# Autodesk Inventor assembly: WedgeBotV1
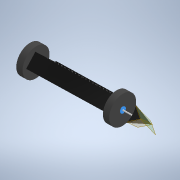
[picture p0: Inventor's stored thumbnail of the model, 180x180]
Saved by Autodesk Inventor 2020 (Build 240168000, 168)
## iProperties
Created: 2023-12-01
Part Number: WedgeBotV1
Document SubType Name: Assembly
Designer: smz3rm
Mass: 451.91 g
Surface Area: 928.874 cm^2
Volume: 362.181 cm^3
Density: 1.24775 g/cm^3
Author: smz3rm
## Documents named in this file (6)
- C:\Users\smz3rm\OneDrive - BP\Documents\DigitalTwin\Models\BattleBot\WedgeBotV1.iam
- C:\Users\smz3rm\OneDrive - BP\Documents\DigitalTwin\Models\BattleBot\DriveMotorV2.ipt
- C:\Users\smz3rm\OneDrive - BP\Documents\DigitalTwin\Models\BattleBot\HubV2.ipt
- C:\Users\smz3rm\OneDrive - BP\Documents\DigitalTwin\Models\BattleBot\WheelV1.ipt
- C:\Users\smz3rm\OneDrive - BP\Documents\DigitalTwin\Models\BattleBot\BodyWedgeV3.ipt
- C:\Users\smz3rm\OneDrive - BP\Documents\DigitalTwin\Models\BattleBot\BatteryV1.ipt
## Components (8 placed, 5 different names)
1. DriveMotorV2:1 — Mate:2, Mate:13, Mate:14, Mate:15
2. HubV2:1 — Cylindrical:1, Mate:1, Mate:2, Mate:21
3. WheelV1:1 — Cylindrical:1, Mate:1, Tangent:1
4. WheelV1:2 — Mate:7, Mate:8
5. DriveMotorV2:2 — Mate:9, Mate:10, Mate:11, Mate:12
6. HubV2:2 — Mate:7, Mate:8, Mate:9, Mate:20
7. BodyWedgeV3:1 — Mate:10, Mate:11, Mate:12, Mate:13, Mate:14, Mate:15, Mate:16, Mate:17, Mate:18, Mate:19, Mate:20, Mate:21
8. BatteryV1:1 — Mate:16, Mate:17, Mate:18
## Relationships (19: Mate 17, CylindricalJoint 1, Tangent 1)
- Cylindrical:1: HubV2:1 ↔ WheelV1:1
- Mate:1: HubV2:1 ↔ WheelV1:1
- Mate:2: DriveMotorV2:1 ↔ HubV2:1
- Mate:7: WheelV1:2 ↔ HubV2:2
- Mate:8: WheelV1:2 ↔ HubV2:2
- Mate:9: DriveMotorV2:2 ↔ HubV2:2
- Mate:10: DriveMotorV2:2 ↔ BodyWedgeV3:1
- Mate:11: DriveMotorV2:2 ↔ BodyWedgeV3:1
- Mate:12: DriveMotorV2:2 ↔ BodyWedgeV3:1
- Mate:13: DriveMotorV2:1 ↔ BodyWedgeV3:1
- Mate:14: DriveMotorV2:1 ↔ BodyWedgeV3:1
- Mate:15: DriveMotorV2:1 ↔ BodyWedgeV3:1
- Mate:16: BodyWedgeV3:1 ↔ BatteryV1:1
- Mate:17: BodyWedgeV3:1 ↔ BatteryV1:1
- Mate:18: BodyWedgeV3:1 ↔ BatteryV1:1
- Mate:19: BodyWedgeV3:1
- Mate:20: HubV2:2 ↔ BodyWedgeV3:1
- Mate:21: HubV2:1 ↔ BodyWedgeV3:1
- Tangent:1: WheelV1:1
